(part 1 of 2)
# Autodesk Inventor assembly: 000 Ensamblaje hw_DAA - PCB FPGA
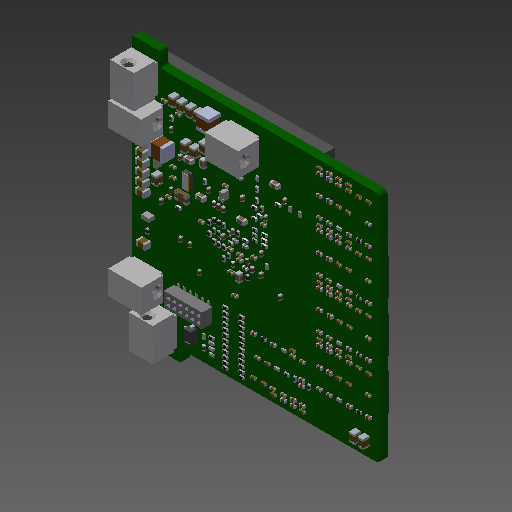
[picture p0: Inventor's stored thumbnail of the model, 512x512]
Saved by Autodesk Inventor 2018 (Build 220112000, 112)
## iProperties
Created: 2024-03-13
Part Number: 000 Ensamblaje hw_DAA - PCB FPGA
Document SubType Name: Assembly
Designer: cda1
Author: cda1
## Documents named in this file (44)
- C:\Users\cda1\Git\DAA\items\hw_DAA\variants\BASIC\3d\000 Ensamblaje hw_DAA - PCB FPGA.iam
- C:\Users\cda1\Git\DAA\items\hw_DAA\3d\hw_DAA - PCB FPGA.ipt
- C:\Users\cda1\Git\DAA\items\_accessories\Componentes PCB\FPGA\3d\3d_Xilinx\XCZU15EG-2FFVB1156I\XCZU15EG-2FFVB1156I.iam
- C:\Users\cda1\Git\DAA\items\_accessories\Componentes PCB\Mosfet\3d_Diodes Inc\3d\DMG1012TQ-7\DMG1012TQ-7.iam
- C:\Users\cda1\Git\DAA\items\_accessories\Componentes PCB\Conectores\3d_Samtec\3d\CLP-106-02-F-D-BE-TR\CLP-106-02-F-D-BE-TR.iam
- C:\Users\cda1\Git\DAA\items\_accessories\Componentes PCB\Capacitadores\3d_Murata Electronics\3d\GRM32EC80E337ME05L\GRM32EC80E337ME05L.ipt
- C:\Users\cda1\Git\DAA\items\_accessories\Componentes PCB\Capacitadores\3d_Murata Electronics\3d\GRT155R61E105KE01D.ipt
- C:\Users\cda1\Git\DAA\items\_accessories\Componentes PCB\Diodos\3d_Semtech\3d\RCLAMP3324PQTCT\RCLAMP3324PQTCT.ipt
- C:\Users\cda1\Git\DAA\items\_accessories\Componentes PCB\Multiplexor\3d_TI\3d\SN74LVC1G08QDCKRQ1.ipt
- C:\Users\cda1\Git\DAA\items\_accessories\Componentes PCB\Resistencias\3d_Panasonic\3d\ERJ-U02F4701X\ERJ-U02F4701X.iam
- C:\Users\cda1\Git\DAA\items\_accessories\Componentes PCB\Resistencias\3d_Panasonic\3d\ERJ-2RKF1002X.ipt
- C:\Users\cda1\Git\DAA\items\_accessories\Componentes PCB\Resistencias\3d_Panasonic\3d\ERJ-2GE0R00X.ipt
- C:\Users\cda1\Git\DAA\items\_accessories\Componentes PCB\Resistencias\3d_Panasonic\3d\ERJ-U02F20R0X\ERJ-U02F20R0X.iam
- C:\Users\cda1\Git\DAA\items\_accessories\Componentes PCB\Capacitadores\3d_TDK\3d\CGA2B3X7R1H104K050BD.ipt
- C:\Users\cda1\Git\DAA\items\_accessories\Componentes PCB\Capacitadores\3d_Murata Electronics\3d\NFM18HC106D0G3L\NFM18HC106D0G3L.ipt
- C:\Users\cda1\Git\DAA\items\_accessories\Componentes PCB\Capacitadores\3d_Murata Electronics\3d\GRM21BC80G107ME15L\GRM21BC80G107ME15L.iam
- C:\Users\cda1\Git\DAA\items\_accessories\Componentes PCB\Capacitadores\3d_TDK\3d\CGA2B1X7S1C474K050BC.ipt
- C:\Users\cda1\Git\DAA\items\_accessories\Componentes PCB\Capacitadores\3d_TDK\3d\CGA2B3X7R1H683K050BB\CGA2B3X7R1H683K050BB.iam
- C:\Users\cda1\Git\DAA\items\_accessories\Componentes PCB\Condensadores\3d-Murata\3d\GRT155C81C225KE13D.ipt
- C:\Users\cda1\Git\DAA\items\_accessories\Componentes PCB\Condensadores\3d-Murata\3d\GRT155R61A475ME13D\GRT155R61A475ME13D.iam
- C:\Users\cda1\Git\DAA\items\_accessories\Componentes PCB\Capacitadores\3d_TDK\3d\CGA2B3X8R1H103K050BB.ipt
- C:\Users\cda1\Git\DAA\items\_accessories\Componentes PCB\Capacitadores\3d_Murata Electronics\3d\GCM1555C1H101JA16D.ipt
- C:\Users\cda1\Git\DAA\items\_accessories\Componentes PCB\Capacitadores\3d_Murata Electronics\3d\GRT155D70G106ME13J\GRT155D70G106ME13J.iam
- C:\Users\cda1\Git\DAA\items\_accessories\Componentes PCB\Capacitadores\3d_Genérico\3d\CAPC-0603-T0.9-BN.ipt
- C:\Users\cda1\Git\DAA\items\_accessories\Componentes PCB\Cristales\3d_ECS\3d\ECS-.327-12.5-34QCS-TR\ECS-.327-12.5-34QCS-TR.ipt
- C:\Users\cda1\Git\DAA\items\_accessories\Componentes PCB\Oscilador\3d_SiTime\SiT8008BI-11-33E-33.333333E\SiT8008BI-11-33E-33.333333E.ipt
- C:\Users\cda1\Git\DAA\items\_accessories\Componentes PCB\Capacitadores\3d_AVX\3d\04025A220C4T2A.ipt
- C:\Users\cda1\Git\DAA\items\_accessories\Componentes PCB\Capacitadores\3d_Genérico\3d\CAPC-0402-T0.55-BN.ipt
- C:\Users\cda1\Git\DAA\items\_accessories\Componentes PCB\Temp Sensor\3d_Texas_Instruments\TMP451HQDQFRQ1\TMP451HQDQFRQ1.iam
- C:\Users\cda1\Git\DAA\items\_accessories\Componentes PCB\Diodos\3d_Diodes Incorporated\3d\BZT52C3V3-7-F.ipt
- C:\Users\cda1\Git\DAA\items\_accessories\Componentes PCB\Resistencias\3d_Vishay\3d\CRCW040239R0FKED\CRCW040239R0FKED.ipt
- C:\Users\cda1\Git\DAA\items\_accessories\Componentes PCB\Resistencias\3d_Vishay\3d\CRCW040249R9FKED\CRCW040249R9FKED.ipt
- C:\Users\cda1\Git\DAA\items\_accessories\Componentes PCB\Resistencias\3d_Vishay\3d\CRCW040236R0FKED\CRCW040236R0FKED.ipt
- C:\Users\cda1\Git\DAA\items\_accessories\Componentes PCB\Resistencias\3d_Panasonic\3d\ERJ-2RKF56R0X\ERJ-2RKF56R0X.iam
- C:\Users\cda1\Git\DAA\items\_accessories\Componentes PCB\Resistencias\3d_Vishay\3d\CRCW0402240RFKED\CRCW0402240RFKED.ipt
- C:\Users\cda1\Git\DAA\items\_accessories\Componentes PCB\Resistencias\3d_Vishay\3d\CRCW0402499RFKEDHP\CRCW0402499RFKEDHP.iam
- C:\Users\cda1\Git\DAA\items\_accessories\Componentes PCB\Resistencias\3d_Panasonic\3d\ERJ-2RKF1001X.ipt
- C:\Users\cda1\Git\DAA\items\_accessories\Componentes PCB\Resistencias\3d_Yageo\3d\RC0402FR-7W100RL\RC0402FR-7W100RL.iam
- C:\Users\cda1\Git\DAA\items\_accessories\Componentes PCB\Ferrita\3d_Murata Electronics\3d\BLM15PX121SH1D\BLM15PX121SH1D.ipt
- C:\Users\cda1\Git\DAA\items\_accessories\Componentes PCB\Resistencias\3d_Genérico\RESC-0402.ipt
- C:\Users\cda1\Git\DAA\items\_accessories\Componentes PCB\Resistencias\3d_Vishay\3d\CRCW04024M70FKED\CRCW04024M70FKED.ipt
- C:\Users\cda1\Git\DAA\items\_accessories\Componentes PCB\Elementos mecanicos soldables\3d_Wurth Electronics\3d\SMD\WP-SMRA Redcube (M2) 7466302.ipt
- C:\Users\cda1\Git\DAA\items\_accessories\Componentes PCB\Elementos mecanicos soldables\3d_Wurth Electronics\3d\SMD\WP-SMRA Redcube (M2) 746630200.ipt
- C:\Users\cda1\Git\DAA\items\_accessories\Componentes PCB\DRAM\MT40A1G16TD-062E_AAT_F\MT40A1G16TD-062E_AAT_F.ipt
## Components (319 placed, 43 different names)
1. hw_DAA - PCB FPGA:1 — Coincidencia:1, Coincidencia:12, Coincidencia:13, Coincidencia:14, Coincidencia:15, Coincidencia:34, Coincidencia:35, Coincidencia:99, Coincidencia:100, Coincidencia:101, Coincidencia:102, Ángulo:6, Coincidencia:103, Ángulo:7, Coincidencia:104, Ángulo:8, Coincidencia:105, Coincidencia:106, Coincidencia:107, Coincidencia:108, Coincidencia:109, Coincidencia:110, Coincidencia:111, Coincidencia:112, Coincidencia:113, Ángulo:9, Coincidencia:114, Coincidencia:115, Coincidencia:116, Ángulo:10, Coincidencia:117, Coincidencia:118, Ángulo:11, Coincidencia:119, Coincidencia:120, Coincidencia:121, Coincidencia:122, Coincidencia:123, Coincidencia:124, Coincidencia:125, Coincidencia:126, Coincidencia:127, Coincidencia:128, Ángulo:12, Coincidencia:129, Ángulo:13, Coincidencia:130, Coincidencia:131, Coincidencia:132, Coincidencia:133, Coincidencia:134, Coincidencia:135, Coincidencia:136, Coincidencia:137, Coincidencia:138, Coincidencia:139, Coincidencia:140, Coincidencia:141, Coincidencia:142, Coincidencia:143, Coincidencia:144, Coincidencia:145, Coincidencia:146, Coincidencia:147, Coincidencia:148, Coincidencia:149, Coincidencia:150, Coincidencia:151, Coincidencia:152, Coincidencia:153, Coincidencia:154, Coincidencia:155, Coincidencia:156, Coincidencia:157, Coincidencia:158, Coincidencia:159, Coincidencia:160, Coincidencia:161, Coincidencia:162, Coincidencia:163, Coincidencia:164, Coincidencia:165, Coincidencia:166, Coincidencia:167, Coincidencia:168, Coincidencia:169, Coincidencia:170, Coincidencia:171, Coincidencia:172, Coincidencia:173, Coincidencia:174, Coincidencia:175, Coincidencia:176, Coincidencia:177, Coincidencia:178, Coincidencia:179, Coincidencia:181, Coincidencia:182, Coincidencia:183, Coincidencia:184, Coincidencia:185, Coincidencia:186, Coincidencia:187, Coincidencia:188, Coincidencia:189, Coincidencia:190, Coincidencia:191, Coincidencia:192, Coincidencia:193, Coincidencia:194, Coincidencia:195, Coincidencia:196, Coincidencia:197, Coincidencia:198, Coincidencia:199, Coincidencia:200, Coincidencia:201, Coincidencia:202, Coincidencia:203, Coincidencia:204, Coincidencia:205, Coincidencia:206, Coincidencia:207, Coincidencia:208, Coincidencia:209, Coincidencia:210, Coincidencia:211, Coincidencia:212, Coincidencia:213, Coincidencia:214, Coincidencia:215, Coincidencia:216, Coincidencia:217, Coincidencia:218, Coincidencia:219, Coincidencia:220, Coincidencia:221, Coincidencia:222, Ángulo:14, Ángulo:15, Coincidencia:223, Coincidencia:224, Coincidencia:225, Coincidencia:226, Coincidencia:227, Coincidencia:228, Coincidencia:229, Coincidencia:230, Coincidencia:231, Coincidencia:232, Coincidencia:233, Coincidencia:234, Coincidencia:235, Coincidencia:236, Coincidencia:237, Coincidencia:238, Coincidencia:239, Coincidencia:240, Coincidencia:241, Coincidencia:251, Coincidencia:252, Coincidencia:253, Coincidencia:254, Coincidencia:255, Ángulo:17, Ángulo:18, Ángulo:19, Coincidencia:256, Coincidencia:257, Coincidencia:258, Ángulo:20, Coincidencia:259, Coincidencia:260, Ángulo:21, Coincidencia:261, Coincidencia:262, Coincidencia:263, Ángulo:22, Coincidencia:264, Ángulo:23, Coincidencia:265, Ángulo:24, Coincidencia:266, Ángulo:25, Coincidencia:267, Coincidencia:268, Coincidencia:269, Ángulo:26, Coincidencia:270, Coincidencia:271, Coincidencia:272, Coincidencia:273, Coincidencia:274, Coincidencia:275, Coincidencia:276, Coincidencia:277, Coincidencia:278, Ángulo:27, Coincidencia:279, Ángulo:28, Coincidencia:280, Ángulo:29, Coincidencia:281, Ángulo:30, Coincidencia:282, Ángulo:31, Coincidencia:283, Ángulo:32, Coincidencia:284, Coincidencia:285, Coincidencia:286, Ángulo:33, Coincidencia:287, Coincidencia:288, Coincidencia:289, Coincidencia:290, Coincidencia:291, Coincidencia:292, Coincidencia:293, Coincidencia:294, Coincidencia:295, Ángulo:34, Coincidencia:296, Ángulo:35, Coincidencia:297, Ángulo:36, Coincidencia:298, Ángulo:37, Coincidencia:299, Coincidencia:300, Ángulo:38, Coincidencia:301, Coincidencia:302, Ángulo:39, Coincidencia:303, Coincidencia:304, Coincidencia:305, Coincidencia:306, Coincidencia:307, Coincidencia:314, Coincidencia:315, Coincidencia:316, Coincidencia:317, Coincidencia:318, Coincidencia:319, Ángulo:40, Coincidencia:320, Coincidencia:321, Ángulo:41, Ángulo:42, Coincidencia:322, Coincidencia:323, Ángulo:43, Ángulo:44, Coincidencia:324, Coincidencia:325, Coincidencia:326, Coincidencia:327, Ángulo:45, Ángulo:46, Coincidencia:328, Coincidencia:329, Coincidencia:330, Coincidencia:331, Coincidencia:332, Coincidencia:333, Ángulo:47, Coincidencia:334, Coincidencia:335, Coincidencia:336, Coincidencia:337, Coincidencia:338, Ángulo:48, Coincidencia:339, Ángulo:49, Coincidencia:340, Coincidencia:341, Ángulo:50, Coincidencia:342, Coincidencia:343, Coincidencia:344, Ángulo:51, Coincidencia:345, Coincidencia:346, Coincidencia:347, Coincidencia:348, Ángulo:52, Coincidencia:349, Coincidencia:350, Ángulo:53, Ángulo:54, Coincidencia:351, Ángulo:55, Coincidencia:352, Coincidencia:353, Coincidencia:354, Ángulo:56, Coincidencia:355, Ángulo:57, Coincidencia:356, Ángulo:58, Coincidencia:357, Coincidencia:358, Ángulo:59, Ángulo:60, Coincidencia:359, Ángulo:61, Coincidencia:360, Coincidencia:361, Ángulo:62, Coincidencia:362, Coincidencia:363, Ángulo:63, Ángulo:64, Coincidencia:364, Ángulo:65, Coincidencia:365, Ángulo:66, Coincidencia:366, Coincidencia:367, Ángulo:67, Coincidencia:368, Ángulo:68, Coincidencia:369, Ángulo:69, Coincidencia:370, Ángulo:70, Coincidencia:371, Coincidencia:372, Coincidencia:373, Coincidencia:374, Coincidencia:375, Coincidencia:376, Coincidencia:377, Coincidencia:378, Coincidencia:379, Ángulo:71, Coincidencia:380, Coincidencia:381, Ángulo:72, Coincidencia:382, Ángulo:73, Coincidencia:384, Ángulo:74, Coincidencia:385, Ángulo:75, Coincidencia:387, Ángulo:76, Coincidencia:388, Nivelación:2, Nivelación:3, Ángulo:77, Ángulo:78, Ángulo:79, Ángulo:80, Ángulo:81, Ángulo:82, Ángulo:83, Ángulo:84, Ángulo:85, Coincidencia:394, Coincidencia:395, Coincidencia:396, Coincidencia:397, Coincidencia:398, Coincidencia:399, Coincidencia:400, Coincidencia:401, Coincidencia:402, Coincidencia:403, Coincidencia:404, Coincidencia:405, Coincidencia:406, Coincidencia:407, Coincidencia:408, Coincidencia:409, Coincidencia:410, Coincidencia:411, Coincidencia:412, Coincidencia:413, Coincidencia:414, Coincidencia:415, Coincidencia:416, Coincidencia:417, Coincidencia:418, Coincidencia:419, Coincidencia:420, Coincidencia:421, Coincidencia:422, Coincidencia:423, Coincidencia:424, Coincidencia:425, Coincidencia:426, Ángulo:86, Coincidencia:428, Nivelación:5, Ángulo:87, Coincidencia:430, Coincidencia:431, Coincidencia:432, Ángulo:88, Ángulo:89
2. XCZU15EG-2FFVB1156I:1 [sub-assembly] — Coincidencia:1
3. DMG1012TQ-7:1 [sub-assembly] — Coincidencia:13, Coincidencia:14, Ángulo:5
4. DMG1012TQ-7:2 [sub-assembly] — Coincidencia:12, Coincidencia:15, Ángulo:5
5. GRM32EC80E337ME05L:1 — Coincidencia:34, Ángulo:12
6. GRM32EC80E337ME05L:2 — Coincidencia:35
7. RCLAMP3324PQTCT:1 — Coincidencia:100
8. RCLAMP3324PQTCT:2 — Coincidencia:99
9. SN74LVC1G08QDCKRQ1:1 — Coincidencia:101, Coincidencia:102, Ángulo:6
10. ERJ-U02F4701X:1 [sub-assembly] — Coincidencia:103, Ángulo:7
11. ERJ-U02F4701X:2 [sub-assembly] — Coincidencia:104, Ángulo:8
12. ERJ-U02F4701X:3 [sub-assembly] — Coincidencia:105
13. ERJ-2RKF1002X:1 — Coincidencia:106
14. ERJ-2GE0R00X:1 — Coincidencia:107
15. ERJ-U02F4701X:4 [sub-assembly] — Coincidencia:108
16. ERJ-U02F4701X:5 [sub-assembly] — Coincidencia:109
17. ERJ-U02F4701X:6 [sub-assembly] — Coincidencia:110
18. ERJ-U02F20R0X:1 [sub-assembly] — Coincidencia:111
19. ERJ-U02F4701X:7 [sub-assembly] — Coincidencia:112
20. ERJ-U02F4701X:8 [sub-assembly] — Coincidencia:113, Ángulo:9
21. CGA2B3X7R1H104K050BD:1 — Coincidencia:114
22. CGA2B3X7R1H104K050BD:2 — Coincidencia:116, Ángulo:10
23. CGA2B3X7R1H104K050BD:3 — Coincidencia:115
24. NFM18HC106D0G3L:1 — Coincidencia:117
25. CGA2B3X7R1H104K050BD:4 — Coincidencia:118, Ángulo:11
26. CGA2B3X7R1H104K050BD:5 — Coincidencia:119
27. CGA2B3X7R1H104K050BD:6 — Coincidencia:120, Ángulo:87
28. GRT155R61E105KE01D:64 — Coincidencia:121
29. GRT155R61E105KE01D:65 — Coincidencia:122
30. CGA2B3X7R1H104K050BD:7 — Coincidencia:123
31. CGA2B3X7R1H104K050BD:8 — Coincidencia:124
32. GRT155R61E105KE01D:66 — Coincidencia:125
33. GRT155R61E105KE01D:67 — Coincidencia:126
34. CGA2B3X7R1H104K050BD:9 — Coincidencia:127
35. CGA2B3X7R1H104K050BD:10 — Coincidencia:128
36. GRM21BC80G107ME15L:1 [sub-assembly] — Coincidencia:129, Ángulo:13
37. GRM21BC80G107ME15L:2 [sub-assembly] — Coincidencia:130
38. GRM21BC80G107ME15L:3 [sub-assembly] — Coincidencia:131
39. GRM21BC80G107ME15L:4 [sub-assembly] — Coincidencia:132
40. GRM21BC80G107ME15L:5 [sub-assembly] — Coincidencia:133
41. GRM21BC80G107ME15L:6 [sub-assembly] — Coincidencia:134
42. GRM21BC80G107ME15L:7 [sub-assembly] — Coincidencia:135
43. GRM21BC80G107ME15L:8 [sub-assembly] — Coincidencia:136
44. GRM21BC80G107ME15L:9 [sub-assembly] — Coincidencia:137
45. GRM21BC80G107ME15L:10 [sub-assembly] — Coincidencia:138
46. GRM21BC80G107ME15L:11 [sub-assembly] — Coincidencia:139
47. GRM21BC80G107ME15L:12 [sub-assembly] — Coincidencia:140
48. GRM21BC80G107ME15L:13 [sub-assembly] — Coincidencia:141
49. GRM21BC80G107ME15L:14 [sub-assembly] — Coincidencia:142
50. GRM21BC80G107ME15L:15 [sub-assembly] — Coincidencia:143
51. CGA2B3X7R1H104K050BD:11 — Coincidencia:145
52. CGA2B3X7R1H104K050BD:12 — Coincidencia:144
53. CGA2B3X7R1H104K050BD:13 — Coincidencia:146
54. CGA2B1X7S1C474K050BC:1 — Coincidencia:147
55. CGA2B3X7R1H683K050BB:1 [sub-assembly] — Coincidencia:148
56. CGA2B1X7S1C474K050BC:2 — Coincidencia:149
57. GRT155R61E105KE01D:68 — Coincidencia:150
58. GRT155C81C225KE13D:1 — Coincidencia:151
59. GRT155R61A475ME13D:1 [sub-assembly] — Coincidencia:152
60. CGA2B3X7R1H104K050BD:14 — Coincidencia:153
61. GRT155R61E105KE01D:69 — Coincidencia:154
62. GRT155C81C225KE13D:2 — Coincidencia:155
63. CGA2B3X7R1H683K050BB:2 [sub-assembly] — Coincidencia:156
64. CGA2B3X7R1H104K050BD:15 — Coincidencia:157
65. GRT155R61A475ME13D:2 [sub-assembly] — Coincidencia:158
66. GRT155R61A475ME13D:3 [sub-assembly] — Coincidencia:159
67. GRT155R61A475ME13D:4 [sub-assembly] — Coincidencia:160
68. GRT155R61E105KE01D:70 — Coincidencia:161
69. GRT155R61E105KE01D:71 — Coincidencia:162
70. CGA2B3X7R1H104K050BD:16 — Coincidencia:163
71. CGA2B1X7S1C474K050BC:3 — Coincidencia:164
72. CGA2B1X7S1C474K050BC:4 — Coincidencia:165
73. CGA2B3X7R1H683K050BB:3 [sub-assembly] — Coincidencia:166
74. GRT155R61E105KE01D:72 — Coincidencia:167
75. GRT155C81C225KE13D:3 — Coincidencia:168
76. GRT155R61A475ME13D:5 [sub-assembly] — Coincidencia:169
77. GRT155R61A475ME13D:6 [sub-assembly] — Coincidencia:170
78. CGA2B3X7R1H104K050BD:17 — Coincidencia:171
79. CGA2B3X7R1H104K050BD:18 — Coincidencia:172
80. GRT155R61E105KE01D:73 — Coincidencia:173
81. GRT155C81C225KE13D:4 — Coincidencia:174
82. CGA2B3X7R1H683K050BB:4 [sub-assembly] — Coincidencia:175
83. CGA2B3X7R1H104K050BD:19 — Coincidencia:176
84. GRT155R61A475ME13D:7 [sub-assembly] — Coincidencia:177
85. GRT155R61A475ME13D:8 [sub-assembly] — Coincidencia:178
86. GRT155R61A475ME13D:9 [sub-assembly] — Coincidencia:179
87. GRT155R61E105KE01D:75 — Coincidencia:181
88. GRT155R61E105KE01D:76 — Coincidencia:182
89. CGA2B3X7R1H104K050BD:20 — Coincidencia:183
90. CGA2B1X7S1C474K050BC:5 — Coincidencia:184
91. CGA2B1X7S1C474K050BC:6 — Coincidencia:185
92. CGA2B3X7R1H683K050BB:5 [sub-assembly] — Coincidencia:186
93. GRT155R61E105KE01D:77 — Coincidencia:187
94. GRT155C81C225KE13D:5 — Coincidencia:188
95. GRT155R61A475ME13D:10 [sub-assembly] — Coincidencia:189
96. GRT155R61A475ME13D:11 [sub-assembly] — Coincidencia:190
97. CGA2B3X7R1H104K050BD:21 — Coincidencia:191
98. CGA2B3X7R1H104K050BD:22 — Coincidencia:192
99. GRT155R61E105KE01D:78 — Coincidencia:193
100. GRT155C81C225KE13D:6 — Coincidencia:194
101. CGA2B3X7R1H683K050BB:6 [sub-assembly] — Coincidencia:195
102. CGA2B3X7R1H104K050BD:23 — Coincidencia:196
103. GRT155R61A475ME13D:12 [sub-assembly] — Coincidencia:197
104. GRT155R61A475ME13D:13 [sub-assembly] — Coincidencia:198
105. GRT155R61A475ME13D:14 [sub-assembly] — Coincidencia:199
106. GRT155R61E105KE01D:79 — Coincidencia:200
107. GRT155R61E105KE01D:80 — Coincidencia:201
108. CGA2B3X7R1H104K050BD:24 — Coincidencia:202
109. CGA2B1X7S1C474K050BC:7 — Coincidencia:203
110. CGA2B1X7S1C474K050BC:8 — Coincidencia:204
111. CGA2B3X7R1H683K050BB:7 [sub-assembly] — Coincidencia:205
112. GRT155R61E105KE01D:81 — Coincidencia:206
113. GRT155C81C225KE13D:7 — Coincidencia:207
114. GRT155R61A475ME13D:15 [sub-assembly] — Coincidencia:208
115. GRT155R61A475ME13D:16 [sub-assembly] — Coincidencia:209
116. CGA2B3X7R1H104K050BD:25 — Coincidencia:210
117. CGA2B3X7R1H104K050BD:26 — Coincidencia:211
118. GRT155R61E105KE01D:82 — Coincidencia:212
119. GRT155C81C225KE13D:8 — Coincidencia:213
120. CGA2B3X7R1H683K050BB:8 [sub-assembly] — Coincidencia:214
121. CGA2B3X7R1H104K050BD:27 — Coincidencia:215
122. GRT155R61A475ME13D:17 [sub-assembly] — Coincidencia:216
123. GRT155R61A475ME13D:18 [sub-assembly] — Coincidencia:217
124. GRT155R61A475ME13D:19 [sub-assembly] — Coincidencia:218
125. GRT155R61E105KE01D:83 — Coincidencia:219
126. GRT155R61E105KE01D:84 — Coincidencia:220
127. GRM21BC80G107ME15L:16 [sub-assembly] — Coincidencia:221, Ángulo:14
128. GRM21BC80G107ME15L:17 [sub-assembly] — Coincidencia:222, Ángulo:15
129. GRT155R61E105KE01D:85 — Coincidencia:223
130. GRT155R61E105KE01D:86 — Coincidencia:224
131. GRT155R61A475ME13D:20 [sub-assembly] — Coincidencia:225
132. GRT155R61A475ME13D:21 [sub-assembly] — Coincidencia:226
133. CGA2B3X7R1H683K050BB:9 [sub-assembly] — Coincidencia:227
134. GRT155R61A475ME13D:22 [sub-assembly] — Coincidencia:228
135. CGA2B3X7R1H104K050BD:28 — Coincidencia:229
136. GRT155C81C225KE13D:9 — Coincidencia:230
137. GRT155R61E105KE01D:87 — Coincidencia:231
138. CGA2B3X7R1H104K050BD:29 — Coincidencia:232
139. CGA2B3X7R1H104K050BD:30 — Coincidencia:233
140. GRT155R61A475ME13D:23 [sub-assembly] — Coincidencia:234
141. GRT155R61A475ME13D:24 [sub-assembly] — Coincidencia:235
142. GRT155C81C225KE13D:10 — Coincidencia:236
143. GRT155R61E105KE01D:88 — Coincidencia:237
144. CGA2B3X7R1H683K050BB:10 [sub-assembly] — Coincidencia:238
145. CGA2B1X7S1C474K050BC:9 — Coincidencia:239
146. CGA2B1X7S1C474K050BC:10 — Coincidencia:240
147. CGA2B3X7R1H104K050BD:31 — Coincidencia:241
148. GRT155R61E105KE01D:89 — Coincidencia:424
149. GRT155R61E105KE01D:90 — Coincidencia:422
150. GRT155R61E105KE01D:91 — Coincidencia:426
151. GRT155R61E105KE01D:92 — Coincidencia:425
152. GRT155R61E105KE01D:93 — Coincidencia:423
153. GRT155R61E105KE01D:94 — Coincidencia:421
154. GRT155R61E105KE01D:95 — Coincidencia:419
155. GRT155R61E105KE01D:96 — Coincidencia:420
156. GRT155R61E105KE01D:97 — Coincidencia:418, Ángulo:86
157. CGA2B3X8R1H103K050BB:1 — Coincidencia:251, Ángulo:84
158. GCM1555C1H101JA16D:1 — Coincidencia:252
159. GRT155R61A475ME13D:25 [sub-assembly] — Coincidencia:253, Ángulo:17
160. GRT155R61A475ME13D:26 [sub-assembly] — Coincidencia:254, Ángulo:18
161. GRT155R61A475ME13D:27 [sub-assembly] — Coincidencia:255, Ángulo:19
162. NFM18HC106D0G3L:2 — Coincidencia:256
163. GRM21BC80G107ME15L:18 [sub-assembly] — Coincidencia:257
164. GRT155D70G106ME13J:1 [sub-assembly] — Coincidencia:258, Ángulo:20
165. GRT155D70G106ME13J:2 [sub-assembly] — Coincidencia:259
166. CGA2B3X7R1H104K050BD:32 — Coincidencia:260, Ángulo:21
167. GRT155D70G106ME13J:3 [sub-assembly] — Coincidencia:261
168. GRT155D70G106ME13J:4 [sub-assembly] — Coincidencia:262
169. NFM18HC106D0G3L:3 — Coincidencia:263, Ángulo:22
170. GRT155D70G106ME13J:5 [sub-assembly] — Coincidencia:264, Ángulo:23
171. CAPC-0603-T0.9-BN:1 — Coincidencia:265, Ángulo:24
172. GRT155R61A475ME13D:28 [sub-assembly] — Coincidencia:266, Ángulo:25
173. GRT155R61A475ME13D:29 [sub-assembly] — Coincidencia:267, Ángulo:82
174. GRT155R61A475ME13D:30 [sub-assembly] — Coincidencia:268, Ángulo:83
175. ECS-.327-12.5-34QCS-TR:1 — Coincidencia:269, Ángulo:26
176. SiT8008BI-11-33E-33.333333E:1 — Coincidencia:270
177. CAPC-0603-T0.9-BN:2 — Coincidencia:271
178. CAPC-0603-T0.9-BN:3 — Coincidencia:272
179. CAPC-0603-T0.9-BN:4 — Coincidencia:273
180. GRT155D70G106ME13J:6 [sub-assembly] — Coincidencia:274
181. GRT155D70G106ME13J:7 [sub-assembly] — Coincidencia:275
182. GRT155D70G106ME13J:8 [sub-assembly] — Coincidencia:276
183. GRT155D70G106ME13J:9 [sub-assembly] — Coincidencia:277
184. GRT155D70G106ME13J:10 [sub-assembly] — Coincidencia:278, Ángulo:27
185. CGA2B3X7R1H104K050BD:33 — Coincidencia:279, Ángulo:28
186. CGA2B1X7S1C474K050BC:11 — Coincidencia:280, Ángulo:29
187. NFM18HC106D0G3L:4 — Coincidencia:281, Ángulo:30
188. GRT155D70G106ME13J:11 [sub-assembly] — Coincidencia:282, Ángulo:31
189. CAPC-0603-T0.9-BN:5 — Coincidencia:283, Ángulo:32
190. CAPC-0603-T0.9-BN:6 — Coincidencia:284
191. GRT155D70G106ME13J:12 [sub-assembly] — Coincidencia:286, Ángulo:33
192. GRT155D70G106ME13J:13 [sub-assembly] — Coincidencia:285
193. GRT155D70G106ME13J:14 [sub-assembly] — Coincidencia:287
194. GRT155D70G106ME13J:15 [sub-assembly] — Coincidencia:288
195. GRT155D70G106ME13J:16 [sub-assembly] — Coincidencia:289
196. GRT155D70G106ME13J:17 [sub-assembly] — Coincidencia:290
197. GRT155D70G106ME13J:18 [sub-assembly] — Coincidencia:291
198. GRT155D70G106ME13J:19 [sub-assembly] — Coincidencia:292
199. 04025A220C4T2A:1 — Coincidencia:293
200. CAPC-0402-T0.55-BN:1 — Coincidencia:294
201. GRT155D70G106ME13J:20 [sub-assembly] — Coincidencia:295, Ángulo:34
202. GRT155D70G106ME13J:21 [sub-assembly] — Coincidencia:296, Ángulo:35
203. CGA2B3X7R1H104K050BD:34 — Coincidencia:297, Ángulo:36
204. CGA2B1X7S1C474K050BC:12 — Coincidencia:298, Ángulo:37
205. GRT155D70G106ME13J:22 [sub-assembly] — Coincidencia:299
206. 04025A220C4T2A:2 — Coincidencia:300, Ángulo:38
207. GRT155D70G106ME13J:23 [sub-assembly] — Coincidencia:301
208. GRT155D70G106ME13J:24 [sub-assembly] — Coincidencia:302, Ángulo:39
209. GRT155D70G106ME13J:25 [sub-assembly] — Coincidencia:303
210. CAPC-0603-T0.9-BN:7 — Coincidencia:304
211. TMP451HQDQFRQ1:1 [sub-assembly] — Coincidencia:305
212. BZT52C3V3-7-F:1 — Coincidencia:306, Coincidencia:307
213. CRCW040239R0FKED:1 — Coincidencia:314
214. CRCW040249R9FKED:1 — Coincidencia:315, Ángulo:85
215. CRCW040249R9FKED:2 — Coincidencia:316
216. CRCW040236R0FKED:1 — Coincidencia:317
217. CRCW040236R0FKED:2 — Coincidencia:318
218. ERJ-2GE0R00X:2 — Coincidencia:319, Ángulo:40
219. ERJ-2RKF56R0X:1 [sub-assembly] — Coincidencia:321, Ángulo:41
220. ERJ-2RKF56R0X:2 [sub-assembly] — Coincidencia:320, Ángulo:42
221. ERJ-U02F4701X:9 [sub-assembly] — Coincidencia:322, Ángulo:43
222. ERJ-U02F4701X:10 [sub-assembly] — Coincidencia:323, Ángulo:44
223. CRCW0402240RFKED:1 — Coincidencia:324
224. ERJ-U02F4701X:11 [sub-assembly] — Coincidencia:325
225. ERJ-U02F4701X:12 [sub-assembly] — Coincidencia:326, Ángulo:45
226. ERJ-U02F4701X:13 [sub-assembly] — Coincidencia:327, Ángulo:46
227. CRCW0402240RFKED:2 — Coincidencia:328
228. CRCW0402499RFKEDHP:1 [sub-assembly] — Coincidencia:329
229. CRCW0402240RFKED:3 — Coincidencia:330
230. CRCW0402499RFKEDHP:2 [sub-assembly] — Coincidencia:331
231. CRCW0402240RFKED:4 — Coincidencia:332
232. CRCW0402499RFKEDHP:3 [sub-assembly] — Coincidencia:333, Ángulo:47
233. CRCW0402240RFKED:5 — Coincidencia:334
234. CRCW0402499RFKEDHP:4 [sub-assembly] — Coincidencia:335
235. CRCW0402240RFKED:6 — Coincidencia:336
236. CRCW0402499RFKEDHP:5 [sub-assembly] — Coincidencia:337
237. CRCW0402240RFKED:7 — Coincidencia:338, Ángulo:48
238. CRCW0402240RFKED:8 — Coincidencia:339, Ángulo:49
239. ERJ-2RKF1001X:1 — Coincidencia:340
240. RC0402FR-7W100RL:1 [sub-assembly] — Coincidencia:341, Ángulo:50
241. RC0402FR-7W100RL:2 [sub-assembly] — Coincidencia:342
242. ERJ-2RKF1001X:2 — Coincidencia:343
243. ERJ-2RKF1001X:3 — Coincidencia:344, Ángulo:51
244. CRCW0402240RFKED:9 — Coincidencia:345
245. CRCW0402240RFKED:10 — Coincidencia:346
246. BLM15PX121SH1D:1 — Coincidencia:348, Ángulo:52
247. BLM15PX121SH1D:2 — Coincidencia:347
248. ERJ-2RKF1001X:4 — Coincidencia:350, Ángulo:54
249. ERJ-2RKF1001X:5 — Coincidencia:349, Ángulo:53
250. RESC-0402:1 — Coincidencia:351, Ángulo:55
251. ERJ-2RKF1001X:6 — Coincidencia:352
252. RESC-0402:2 — Coincidencia:353
253. CRCW0402240RFKED:11 — Coincidencia:354, Ángulo:56
254. ERJ-U02F4701X:14 [sub-assembly] — Coincidencia:355, Ángulo:57
255. CAPC-0603-T0.9-BN:8 — Coincidencia:356, Ángulo:58
256. CRCW0402499RFKEDHP:6 [sub-assembly] — Coincidencia:357, Ángulo:59
257. CRCW0402499RFKEDHP:7 [sub-assembly] — Coincidencia:358, Ángulo:60
258. ERJ-U02F4701X:15 [sub-assembly] — Coincidencia:359, Ángulo:61
259. ERJ-U02F4701X:16 [sub-assembly] — Coincidencia:360
260. RESC-0402:3 — Coincidencia:361, Ángulo:62
261. ERJ-U02F4701X:17 [sub-assembly] — Coincidencia:362, Ángulo:63
262. ERJ-U02F4701X:18 [sub-assembly] — Coincidencia:363, Ángulo:64
263. RESC-0402:4 — Coincidencia:364, Ángulo:65
264. RESC-0402:5 — Coincidencia:365, Ángulo:66
265. RESC-0402:6 — Coincidencia:366
266. ERJ-U02F4701X:19 [sub-assembly] — Coincidencia:367, Ángulo:67
267. ERJ-U02F4701X:20 [sub-assembly] — Coincidencia:368, Ángulo:68
268. CRCW04024M70FKED:1 — Coincidencia:369, Ángulo:69
269. ERJ-U02F4701X:21 [sub-assembly] — Coincidencia:370, Ángulo:70
270. ERJ-2GE0R00X:3 — Coincidencia:371
271. ERJ-U02F4701X:22 [sub-assembly] — Coincidencia:372
272. RESC-0402:7 — Coincidencia:373
273. RESC-0402:8 — Coincidencia:374
274. ERJ-U02F4701X:23 [sub-assembly] — Coincidencia:375
275. ERJ-U02F4701X:24 [sub-assembly] — Coincidencia:376
276. RESC-0402:9 — Coincidencia:377
277. ERJ-U02F4701X:25 [sub-assembly] — Coincidencia:378
278. CRCW0402499RFKEDHP:8 [sub-assembly] — Coincidencia:379, Ángulo:71
279. BLM15PX121SH1D:3 — Coincidencia:381, Ángulo:72
280. BLM15PX121SH1D:4 — Coincidencia:380
281. CRCW0402240RFKED:12 — Coincidencia:382, Ángulo:73
282. WP-SMRA Redcube (M2) 746630200:2
283. WP-SMRA Redcube (M2) 7466302:2 — Coincidencia:384, Ángulo:74, Nivelación:3
284. WP-SMRA Redcube (M2) 7466302:3 — Coincidencia:385, Ángulo:75, Nivelación:2, Coincidencia:428
285. WP-SMRA Redcube (M2) 746630200:3
286. WP-SMRA Redcube (M2) 746630200:1 — Coincidencia:387, Ángulo:76, Nivelación:5
287. CLP-106-02-F-D-BE-TR:2 [sub-assembly] — Coincidencia:388
288. MT40A1G16TD-062E_AAT_F:1 — Ángulo:81
289. MT40A1G16TD-062E_AAT_F:2 — Ángulo:80
290. MT40A1G16TD-062E_AAT_F:3 — Ángulo:79
291. MT40A1G16TD-062E_AAT_F:4 — Ángulo:78
292. MT40A1G16TD-062E_AAT_F:5 — Ángulo:77
293. CRCW040239R0FKED:2 — Coincidencia:394
294. CRCW040239R0FKED:3 — Coincidencia:395
295. CRCW040239R0FKED:4 — Coincidencia:396
296. CRCW040239R0FKED:5 — Coincidencia:397
297. CRCW040239R0FKED:6 — Coincidencia:398
298. CRCW040239R0FKED:7 — Coincidencia:399
299. CRCW040239R0FKED:8 — Coincidencia:400
300. CRCW040239R0FKED:9 — Coincidencia:401
301. CRCW040239R0FKED:10 — Coincidencia:402
302. CRCW040239R0FKED:11 — Coincidencia:403
303. CRCW040239R0FKED:12 — Coincidencia:404
304. CRCW040239R0FKED:13 — Coincidencia:405
305. CRCW040239R0FKED:14 — Coincidencia:406
306. CRCW040239R0FKED:15 — Coincidencia:407
307. CRCW040239R0FKED:16 — Coincidencia:408
308. CRCW040239R0FKED:17 — Coincidencia:409
309. CRCW040239R0FKED:18 — Coincidencia:410
310. CRCW040239R0FKED:19 — Coincidencia:411
311. CRCW040239R0FKED:20 — Coincidencia:412
312. CRCW040239R0FKED:21 — Coincidencia:413
313. CRCW040239R0FKED:22 — Coincidencia:414
314. CRCW040239R0FKED:23 — Coincidencia:415
315. CRCW040239R0FKED:24 — Coincidencia:416
316. CRCW040239R0FKED:25 — Coincidencia:417
317. ERJ-2RKF1001X:7 — Coincidencia:430
318. ERJ-2RKF1002X:2 — Coincidencia:431, Ángulo:89
319. ERJ-2RKF1002X:3 — Coincidencia:432, Ángulo:88
## Relationships (409: Mate 320, Angle 84, Flush 5)
- Coincidencia:1 [Mate] (0.6 mm): hw_DAA - PCB FPGA:1 ↔ XCZU15EG-2FFVB1156I:1
- Coincidencia:12 [Mate]: hw_DAA - PCB FPGA:1 ↔ DMG1012TQ-7:2
- Coincidencia:13 [Mate]: hw_DAA - PCB FPGA:1 ↔ DMG1012TQ-7:1
- Coincidencia:14 [Mate]: hw_DAA - PCB FPGA:1 ↔ DMG1012TQ-7:1
- Coincidencia:15 [Mate]: hw_DAA - PCB FPGA:1 ↔ DMG1012TQ-7:2
- Coincidencia:34 [Mate]: hw_DAA - PCB FPGA:1 ↔ GRM32EC80E337ME05L:1
- Coincidencia:35 [Mate]: hw_DAA - PCB FPGA:1 ↔ GRM32EC80E337ME05L:2
- Ángulo:5 [Angle] (0 deg): DMG1012TQ-7:1 ↔ DMG1012TQ-7:2
- Coincidencia:99 [Mate]: hw_DAA - PCB FPGA:1 ↔ RCLAMP3324PQTCT:2
- Coincidencia:100 [Mate]: hw_DAA - PCB FPGA:1 ↔ RCLAMP3324PQTCT:1
- Coincidencia:101 [Mate]: hw_DAA - PCB FPGA:1 ↔ SN74LVC1G08QDCKRQ1:1
- Coincidencia:102 [Mate]: hw_DAA - PCB FPGA:1 ↔ SN74LVC1G08QDCKRQ1:1
- Ángulo:6 [Angle] (0 deg): hw_DAA - PCB FPGA:1 ↔ SN74LVC1G08QDCKRQ1:1
- Coincidencia:103 [Mate]: hw_DAA - PCB FPGA:1 ↔ ERJ-U02F4701X:1
- Ángulo:7 [Angle] (0 deg): hw_DAA - PCB FPGA:1 ↔ ERJ-U02F4701X:1
- Coincidencia:104 [Mate]: hw_DAA - PCB FPGA:1 ↔ ERJ-U02F4701X:2
- Ángulo:8 [Angle] (90 deg): hw_DAA - PCB FPGA:1 ↔ ERJ-U02F4701X:2
- Coincidencia:105 [Mate]: hw_DAA - PCB FPGA:1 ↔ ERJ-U02F4701X:3
- Coincidencia:106 [Mate]: hw_DAA - PCB FPGA:1 ↔ ERJ-2RKF1002X:1
- Coincidencia:107 [Mate]: hw_DAA - PCB FPGA:1 ↔ ERJ-2GE0R00X:1
- Coincidencia:108 [Mate]: hw_DAA - PCB FPGA:1 ↔ ERJ-U02F4701X:4
- Coincidencia:109 [Mate]: hw_DAA - PCB FPGA:1 ↔ ERJ-U02F4701X:5
- Coincidencia:110 [Mate]: hw_DAA - PCB FPGA:1 ↔ ERJ-U02F4701X:6
- Coincidencia:111 [Mate]: hw_DAA - PCB FPGA:1 ↔ ERJ-U02F20R0X:1
- Coincidencia:112 [Mate]: hw_DAA - PCB FPGA:1 ↔ ERJ-U02F4701X:7
- Coincidencia:113 [Mate]: hw_DAA - PCB FPGA:1 ↔ ERJ-U02F4701X:8
- Ángulo:9 [Angle] (0 deg): hw_DAA - PCB FPGA:1 ↔ ERJ-U02F4701X:8
- Coincidencia:114 [Mate]: hw_DAA - PCB FPGA:1 ↔ CGA2B3X7R1H104K050BD:1
- Coincidencia:115 [Mate]: hw_DAA - PCB FPGA:1 ↔ CGA2B3X7R1H104K050BD:3
- Coincidencia:116 [Mate]: hw_DAA - PCB FPGA:1 ↔ CGA2B3X7R1H104K050BD:2
- Ángulo:10 [Angle] (0 deg): hw_DAA - PCB FPGA:1 ↔ CGA2B3X7R1H104K050BD:2
- Coincidencia:117 [Mate]: hw_DAA - PCB FPGA:1 ↔ NFM18HC106D0G3L:1
- Coincidencia:118 [Mate]: hw_DAA - PCB FPGA:1 ↔ CGA2B3X7R1H104K050BD:4
- Ángulo:11 [Angle] (0 deg): hw_DAA - PCB FPGA:1 ↔ CGA2B3X7R1H104K050BD:4
- Coincidencia:119 [Mate]: hw_DAA - PCB FPGA:1 ↔ CGA2B3X7R1H104K050BD:5
- Coincidencia:120 [Mate]: hw_DAA - PCB FPGA:1 ↔ CGA2B3X7R1H104K050BD:6
- Coincidencia:121 [Mate]: hw_DAA - PCB FPGA:1 ↔ GRT155R61E105KE01D:64
- Coincidencia:122 [Mate]: hw_DAA - PCB FPGA:1 ↔ GRT155R61E105KE01D:65
- Coincidencia:123 [Mate]: hw_DAA - PCB FPGA:1 ↔ CGA2B3X7R1H104K050BD:7
- Coincidencia:124 [Mate]: hw_DAA - PCB FPGA:1 ↔ CGA2B3X7R1H104K050BD:8
- Coincidencia:125 [Mate]: hw_DAA - PCB FPGA:1 ↔ GRT155R61E105KE01D:66
- Coincidencia:126 [Mate]: hw_DAA - PCB FPGA:1 ↔ GRT155R61E105KE01D:67
- Coincidencia:127 [Mate]: hw_DAA - PCB FPGA:1 ↔ CGA2B3X7R1H104K050BD:9
- Coincidencia:128 [Mate]: hw_DAA - PCB FPGA:1 ↔ CGA2B3X7R1H104K050BD:10
- Ángulo:12 [Angle] (0 deg): hw_DAA - PCB FPGA:1 ↔ GRM32EC80E337ME05L:1
- Coincidencia:129 [Mate]: hw_DAA - PCB FPGA:1 ↔ GRM21BC80G107ME15L:1
- Ángulo:13 [Angle] (0 deg): hw_DAA - PCB FPGA:1 ↔ GRM21BC80G107ME15L:1
- Coincidencia:130 [Mate]: hw_DAA - PCB FPGA:1 ↔ GRM21BC80G107ME15L:2
- Coincidencia:131 [Mate]: hw_DAA - PCB FPGA:1 ↔ GRM21BC80G107ME15L:3
- Coincidencia:132 [Mate]: hw_DAA - PCB FPGA:1 ↔ GRM21BC80G107ME15L:4
- Coincidencia:133 [Mate]: hw_DAA - PCB FPGA:1 ↔ GRM21BC80G107ME15L:5
- Coincidencia:134 [Mate]: hw_DAA - PCB FPGA:1 ↔ GRM21BC80G107ME15L:6
- Coincidencia:135 [Mate]: hw_DAA - PCB FPGA:1 ↔ GRM21BC80G107ME15L:7
- Coincidencia:136 [Mate]: hw_DAA - PCB FPGA:1 ↔ GRM21BC80G107ME15L:8
- Coincidencia:137 [Mate]: hw_DAA - PCB FPGA:1 ↔ GRM21BC80G107ME15L:9
- Coincidencia:138 [Mate]: hw_DAA - PCB FPGA:1 ↔ GRM21BC80G107ME15L:10
- Coincidencia:139 [Mate]: hw_DAA - PCB FPGA:1 ↔ GRM21BC80G107ME15L:11
- Coincidencia:140 [Mate]: hw_DAA - PCB FPGA:1 ↔ GRM21BC80G107ME15L:12
- Coincidencia:141 [Mate]: hw_DAA - PCB FPGA:1 ↔ GRM21BC80G107ME15L:13
- Coincidencia:142 [Mate]: hw_DAA - PCB FPGA:1 ↔ GRM21BC80G107ME15L:14
- Coincidencia:143 [Mate]: hw_DAA - PCB FPGA:1 ↔ GRM21BC80G107ME15L:15
- Coincidencia:144 [Mate]: hw_DAA - PCB FPGA:1 ↔ CGA2B3X7R1H104K050BD:12
- Coincidencia:145 [Mate]: hw_DAA - PCB FPGA:1 ↔ CGA2B3X7R1H104K050BD:11
- Coincidencia:146 [Mate]: hw_DAA - PCB FPGA:1 ↔ CGA2B3X7R1H104K050BD:13
- Coincidencia:147 [Mate]: hw_DAA - PCB FPGA:1 ↔ CGA2B1X7S1C474K050BC:1
- Coincidencia:148 [Mate]: hw_DAA - PCB FPGA:1 ↔ CGA2B3X7R1H683K050BB:1
- Coincidencia:149 [Mate]: hw_DAA - PCB FPGA:1 ↔ CGA2B1X7S1C474K050BC:2
- Coincidencia:150 [Mate]: hw_DAA - PCB FPGA:1 ↔ GRT155R61E105KE01D:68
- Coincidencia:151 [Mate]: hw_DAA - PCB FPGA:1 ↔ GRT155C81C225KE13D:1
- Coincidencia:152 [Mate]: hw_DAA - PCB FPGA:1 ↔ GRT155R61A475ME13D:1
- Coincidencia:153 [Mate]: hw_DAA - PCB FPGA:1 ↔ CGA2B3X7R1H104K050BD:14
- Coincidencia:154 [Mate]: hw_DAA - PCB FPGA:1 ↔ GRT155R61E105KE01D:69
- Coincidencia:155 [Mate]: hw_DAA - PCB FPGA:1 ↔ GRT155C81C225KE13D:2
- Coincidencia:156 [Mate]: hw_DAA - PCB FPGA:1 ↔ CGA2B3X7R1H683K050BB:2
- Coincidencia:157 [Mate]: hw_DAA - PCB FPGA:1 ↔ CGA2B3X7R1H104K050BD:15
- Coincidencia:158 [Mate]: hw_DAA - PCB FPGA:1 ↔ GRT155R61A475ME13D:2
- Coincidencia:159 [Mate]: hw_DAA - PCB FPGA:1 ↔ GRT155R61A475ME13D:3
- Coincidencia:160 [Mate]: hw_DAA - PCB FPGA:1 ↔ GRT155R61A475ME13D:4
- Coincidencia:161 [Mate]: hw_DAA - PCB FPGA:1 ↔ GRT155R61E105KE01D:70
- Coincidencia:162 [Mate]: hw_DAA - PCB FPGA:1 ↔ GRT155R61E105KE01D:71
- Coincidencia:163 [Mate]: hw_DAA - PCB FPGA:1 ↔ CGA2B3X7R1H104K050BD:16
- Coincidencia:164 [Mate]: hw_DAA - PCB FPGA:1 ↔ CGA2B1X7S1C474K050BC:3
- Coincidencia:165 [Mate]: hw_DAA - PCB FPGA:1 ↔ CGA2B1X7S1C474K050BC:4
- Coincidencia:166 [Mate]: hw_DAA - PCB FPGA:1 ↔ CGA2B3X7R1H683K050BB:3
- Coincidencia:167 [Mate]: hw_DAA - PCB FPGA:1 ↔ GRT155R61E105KE01D:72
- Coincidencia:168 [Mate]: hw_DAA - PCB FPGA:1 ↔ GRT155C81C225KE13D:3
- Coincidencia:169 [Mate]: hw_DAA - PCB FPGA:1 ↔ GRT155R61A475ME13D:5
- Coincidencia:170 [Mate]: hw_DAA - PCB FPGA:1 ↔ GRT155R61A475ME13D:6
- Coincidencia:171 [Mate]: hw_DAA - PCB FPGA:1 ↔ CGA2B3X7R1H104K050BD:17
- Coincidencia:172 [Mate]: hw_DAA - PCB FPGA:1 ↔ CGA2B3X7R1H104K050BD:18
- Coincidencia:173 [Mate]: hw_DAA - PCB FPGA:1 ↔ GRT155R61E105KE01D:73
- Coincidencia:174 [Mate]: hw_DAA - PCB FPGA:1 ↔ GRT155C81C225KE13D:4
- Coincidencia:175 [Mate]: hw_DAA - PCB FPGA:1 ↔ CGA2B3X7R1H683K050BB:4
- Coincidencia:176 [Mate]: hw_DAA - PCB FPGA:1 ↔ CGA2B3X7R1H104K050BD:19
- Coincidencia:177 [Mate]: hw_DAA - PCB FPGA:1 ↔ GRT155R61A475ME13D:7
- Coincidencia:178 [Mate]: hw_DAA - PCB FPGA:1 ↔ GRT155R61A475ME13D:8
- Coincidencia:179 [Mate]: hw_DAA - PCB FPGA:1 ↔ GRT155R61A475ME13D:9
- Coincidencia:181 [Mate]: hw_DAA - PCB FPGA:1 ↔ GRT155R61E105KE01D:75
- Coincidencia:182 [Mate]: hw_DAA - PCB FPGA:1 ↔ GRT155R61E105KE01D:76
- Coincidencia:183 [Mate]: hw_DAA - PCB FPGA:1 ↔ CGA2B3X7R1H104K050BD:20
- Coincidencia:184 [Mate]: hw_DAA - PCB FPGA:1 ↔ CGA2B1X7S1C474K050BC:5
- Coincidencia:185 [Mate]: hw_DAA - PCB FPGA:1 ↔ CGA2B1X7S1C474K050BC:6
- Coincidencia:186 [Mate]: hw_DAA - PCB FPGA:1 ↔ CGA2B3X7R1H683K050BB:5
- Coincidencia:187 [Mate]: hw_DAA - PCB FPGA:1 ↔ GRT155R61E105KE01D:77
- Coincidencia:188 [Mate]: hw_DAA - PCB FPGA:1 ↔ GRT155C81C225KE13D:5
- Coincidencia:189 [Mate]: hw_DAA - PCB FPGA:1 ↔ GRT155R61A475ME13D:10
- Coincidencia:190 [Mate]: hw_DAA - PCB FPGA:1 ↔ GRT155R61A475ME13D:11
- Coincidencia:191 [Mate]: hw_DAA - PCB FPGA:1 ↔ CGA2B3X7R1H104K050BD:21
- Coincidencia:192 [Mate]: hw_DAA - PCB FPGA:1 ↔ CGA2B3X7R1H104K050BD:22
- Coincidencia:193 [Mate]: hw_DAA - PCB FPGA:1 ↔ GRT155R61E105KE01D:78
- Coincidencia:194 [Mate]: hw_DAA - PCB FPGA:1 ↔ GRT155C81C225KE13D:6
- Coincidencia:195 [Mate]: hw_DAA - PCB FPGA:1 ↔ CGA2B3X7R1H683K050BB:6
- Coincidencia:196 [Mate]: hw_DAA - PCB FPGA:1 ↔ CGA2B3X7R1H104K050BD:23
- Coincidencia:197 [Mate]: hw_DAA - PCB FPGA:1 ↔ GRT155R61A475ME13D:12
- Coincidencia:198 [Mate]: hw_DAA - PCB FPGA:1 ↔ GRT155R61A475ME13D:13
- Coincidencia:199 [Mate]: hw_DAA - PCB FPGA:1 ↔ GRT155R61A475ME13D:14
- Coincidencia:200 [Mate]: hw_DAA - PCB FPGA:1 ↔ GRT155R61E105KE01D:79
- Coincidencia:201 [Mate]: hw_DAA - PCB FPGA:1 ↔ GRT155R61E105KE01D:80
- Coincidencia:202 [Mate]: hw_DAA - PCB FPGA:1 ↔ CGA2B3X7R1H104K050BD:24
- Coincidencia:203 [Mate]: hw_DAA - PCB FPGA:1 ↔ CGA2B1X7S1C474K050BC:7
- Coincidencia:204 [Mate]: hw_DAA - PCB FPGA:1 ↔ CGA2B1X7S1C474K050BC:8
- Coincidencia:205 [Mate]: hw_DAA - PCB FPGA:1 ↔ CGA2B3X7R1H683K050BB:7